# Autodesk Inventor assembly: 9P Sprocket
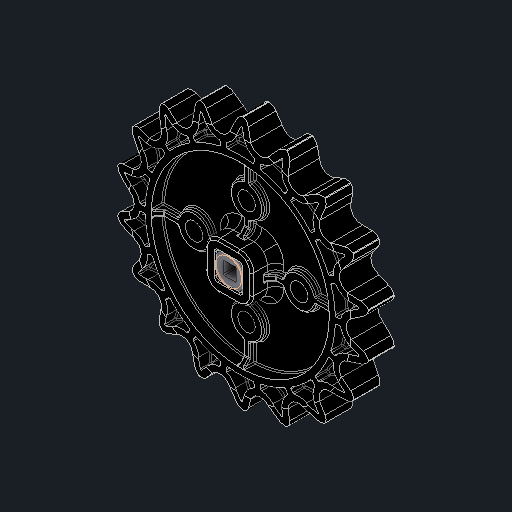
[picture p0: Inventor's stored thumbnail of the model, 512x512]
Saved by Autodesk Inventor 2025 (Build 290162000, 162)
## iProperties
Created: 2022-08-02
Part Number: 9P Sprocket
Document SubType Name: Assembly
Designer: ylu12
Author: ylu12
## Documents named in this file (4)
- D:\VEX\High Stakes\CAD\ROBOPROS-CAD-Inventor\Motion\Sprockets\9P Sprocket\9P 18T Sprocket, Square.iam
- D:\VEX\High Stakes\CAD\ROBOPROS-CAD-Inventor\Motion\HS Shaft Adapter Square.ipt
- D:\VEX\High Stakes\CAD\ROBOPROS-CAD-Inventor\Motion\Sprockets\Reference Files\9P 18T Sprocket, No Insert.ipt
- D:\VEX\High Stakes\CAD\ROBOPROS-CAD-Inventor\Motion\Sprockets\9P Sprocket.iam
## Components (2 placed, 2 different names)
1. Square — Mate:3, Mate:4, Flush:2
2. 18T — Flush:5, Mate:9, Mate:10
## Relationships (6: Mate 4, Flush 2)
- Mate:3: Square
- Mate:4: Square
- Flush:2 (6.35 mm): Square
- Flush:5: 18T
- Mate:9: 18T
- Mate:10: 18T
